# Autodesk Inventor assembly: Arm_right_v3
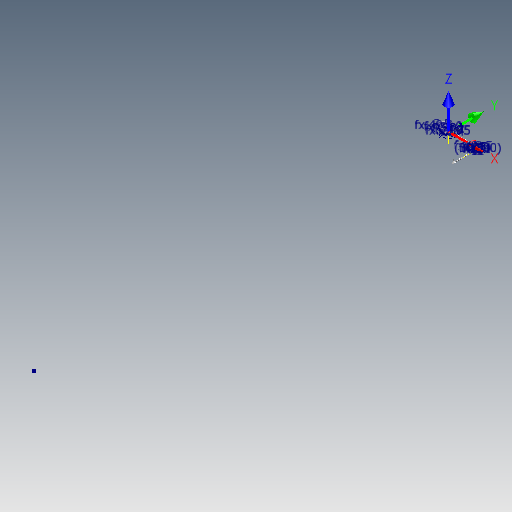
[picture p0: Inventor's stored thumbnail of the model, 512x512]
Saved by Autodesk Inventor 2021.4 (Build 254397000, 397)
## iProperties
Created: 2022-07-06
Part Number: Arm_right_v3
Material: Generisch
Document SubType Name: Assembly
Designer: alexw
Mass: 655.07 g
Surface Area: 1152.93 cm^2
Volume: 246.284 cm^3
Density: 2.65982 g/cm^3
Author: alexw
## Documents named in this file (6)
- C:\Users\alexw\Documents\Inventor\Projects\03_CurrentProjects\MasterThesis\TrainingConsol_220422\Workgroups\Workgroup\Arm_right_v3.iam
- C:\Users\alexw\Documents\Inventor\Projects\03_CurrentProjects\MasterThesis\TrainingConsol_220422\Workgroups\Workgroup\Upper_Arm_v2_Assembly.iam
- C:\Users\alexw\Documents\Inventor\Projects\03_CurrentProjects\MasterThesis\TrainingConsol_220422\Workgroups\Workgroup\Lower_Arm_v3_Assembly.iam
- C:\Users\alexw\Documents\Inventor\Projects\03_CurrentProjects\MasterThesis\TrainingConsol_220422\Workgroups\Workgroup\PTFE_Anlaufscheibe.ipt
- C:\Users\alexw\Documents\Inventor\Projects\03_CurrentProjects\MasterThesis\TrainingConsol_220422\Workgroups\Workgroup\ShoulderJoint_Concept1_LightWeight_Assembly.iam
- C:\Users\alexw\Documents\Inventor\Projects\03_CurrentProjects\MasterThesis\TrainingConsol_220422\Workgroups\Workgroup\ContentCenter\en-US\ISO 7089\ISO 7089 - 4 - 140 HV(1).ipt
## Components (5 placed, 5 different names)
1. ShoulderJoint_Concept1_LightWeight_Assembly:1 [sub-assembly] — Mate:1, Mate:2, Angle:2, Mate:20, Flush:1, Angle:3
2. Upper_Arm_v2_Assembly:1 [sub-assembly] — Mate:1, Mate:2, Mate:3, Mate:4, Mate:5, Mate:6, Mate:7, Mate:8, Mate:12, Angle:1, Angle:2
3. Lower_Arm_v3_Assembly:1 [sub-assembly] — Mate:3, Mate:4, Mate:5, Angle:1
4. PTFE_Anlaufscheibe:1 — Mate:6, Mate:7
5. ISO 7089 4:1 — Mate:8, Mate:12
## Relationships (14: Mate 10, Angle 3, Flush 1)
- Mate:1: ShoulderJoint_Concept1_LightWeight_Assembly:1 ↔ Upper_Arm_v2_Assembly:1
- Mate:2: ShoulderJoint_Concept1_LightWeight_Assembly:1 ↔ Upper_Arm_v2_Assembly:1
- Mate:3: Upper_Arm_v2_Assembly:1 ↔ Lower_Arm_v3_Assembly:1
- Mate:4: Upper_Arm_v2_Assembly:1 ↔ Lower_Arm_v3_Assembly:1
- Mate:5: Upper_Arm_v2_Assembly:1 ↔ Lower_Arm_v3_Assembly:1
- Mate:6: Upper_Arm_v2_Assembly:1 ↔ PTFE_Anlaufscheibe:1
- Mate:7: Upper_Arm_v2_Assembly:1 ↔ PTFE_Anlaufscheibe:1
- Mate:8: Upper_Arm_v2_Assembly:1 ↔ ISO 7089 4:1
- Mate:12: Upper_Arm_v2_Assembly:1 ↔ ISO 7089 4:1
- Angle:1 (-90 deg): Upper_Arm_v2_Assembly:1 ↔ Lower_Arm_v3_Assembly:1
- Angle:2 (0 deg): ShoulderJoint_Concept1_LightWeight_Assembly:1 ↔ Upper_Arm_v2_Assembly:1
- Mate:20: ShoulderJoint_Concept1_LightWeight_Assembly:1
- Flush:1: ShoulderJoint_Concept1_LightWeight_Assembly:1
- Angle:3 (0 deg): ShoulderJoint_Concept1_LightWeight_Assembly:1
